# Autodesk Inventor assembly: Assembly
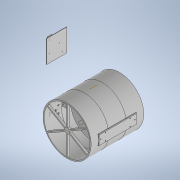
[picture p0: Inventor's stored thumbnail of the model, 180x180]
Saved by Autodesk Inventor 2020.2 (Build 242310000, 310)
## iProperties
Created: 2020-04-12
Part Number: Assembly
Document SubType Name: Assembly
Designer: Josiah
Author: Josiah
## Documents named in this file (9)
- C:\Users\josia\OneDrive\Apps\0011_VentControlValve\Assembly.iam
- C:\Users\josia\OneDrive\Apps\0011_VentControlValve\Base.ipt
- C:\Users\josia\OneDrive\Apps\0011_VentControlValve\center Section Top Half.ipt
- C:\Users\josia\OneDrive\Apps\0011_VentControlValve\Butterfly Valve.ipt
- C:\Users\josia\OneDrive\Apps\0011_VentControlValve\limitSwitch.ipt
- C:\Users\josia\OneDrive\Apps\0011_VentControlValve\motor+Gearbox.ipt
- C:\Users\josia\OneDrive\Apps\0011_VentControlValve\RaspberryPiZeroW.ipt
- C:\Users\josia\OneDrive\Apps\0011_VentControlValve\Electrical Box.ipt
- C:\Users\josia\OneDrive\Apps\0011_VentControlValve\Dual Relay w Breakout Board.ipt
## Components (10 placed, 8 different names)
1. center Section Top Half:1 — Mate:3, Mate:4, Flush:2, Flush:3, Mate:6, Mate:7, Flush:4, Flush:5, Mate:8, Rotational:1, Mate:9, Mate:10, Angle:1, Mate:12, Flush:6
2. Butterfly Valve:1 — Flush:2, Rotational:1, Mate:11
3. Base:1 — Mate:3, Mate:4
4. limitSwitch:1 — Flush:4, Flush:5, Mate:8
5. motor+Gearbox:1 — Mate:11, Angle:1, Mate:12
6. limitSwitch:2 — Flush:3, Mate:6, Mate:7
7. Base:2 — Mate:9, Mate:10
8. RaspberryPiZeroW:1 — Mate:13
9. Electrical Box:1 — Flush:6, Mate:13, Flush:7
10. Dual Relay w Breakout Board:1 — Flush:7
## Relationships (18: Mate 10, Flush 6, RevoluteJoint 1, Angle 1)
- Mate:3: center Section Top Half:1 ↔ Base:1
- Mate:4: center Section Top Half:1 ↔ Base:1
- Flush:2 (5 mm): center Section Top Half:1 ↔ Butterfly Valve:1
- Flush:3: center Section Top Half:1 ↔ limitSwitch:2
- Mate:6 (0.4 mm): center Section Top Half:1 ↔ limitSwitch:2
- Mate:7 (0.4 mm): center Section Top Half:1 ↔ limitSwitch:2
- Flush:4: center Section Top Half:1 ↔ limitSwitch:1
- Flush:5: center Section Top Half:1 ↔ limitSwitch:1
- Mate:8 (0.2 mm): center Section Top Half:1 ↔ limitSwitch:1
- Rotational:1 [RevoluteJoint]: center Section Top Half:1 ↔ Butterfly Valve:1
- Mate:9: center Section Top Half:1 ↔ Base:2
- Mate:10: center Section Top Half:1 ↔ Base:2
- Mate:11: Butterfly Valve:1 ↔ motor+Gearbox:1
- Angle:1 (0 deg): center Section Top Half:1 ↔ motor+Gearbox:1
- Mate:12: center Section Top Half:1 ↔ motor+Gearbox:1
- Flush:6: center Section Top Half:1 ↔ Electrical Box:1
- Mate:13: RaspberryPiZeroW:1 ↔ Electrical Box:1
- Flush:7: Electrical Box:1 ↔ Dual Relay w Breakout Board:1
## Named parameters: outerRadius = 215 mm
